# Autodesk Inventor assembly: ЛЦМК000002.00.05.00.00.00 Компактный вариант крепления
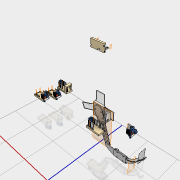
[picture p0: Inventor's stored thumbnail of the model, 180x180]
Saved by Autodesk Inventor 2021.2 (Build 252289000, 289)
## iProperties
Created: 2025-11-11
Part Number: ЛЦМК000002.00.05.00.00.00 Компактный вариант крепления
Document SubType Name: Assembly
Designer: Захаров
Author: Захаров
## Documents named in this file (17)
- C:\Users\User\Documents\CaseARHead1\ЛЦМК000002.00.05.00.00.00 Компактный вариант крепления.iam
- ЛЦМК000002.00.03.00.00.00 Облегченный вариант крепления.iam
- C:\Users\User\Documents\CaseARHead1\ЛЦМК000002.00.00.00.00.08-01.ipt
- C:\Users\User\Documents\CaseARHead1\ЛЦМК000002.00.00.00.00.15.ipt
- C:\Users\User\Documents\CaseARHead1\ЛЦМК000002.00.00.00.00.18-01.ipt
- C:\Users\User\Documents\CaseARHead1\ЛЦМК000002.00.00.00.00.19 мост.ipt
- C:\Users\User\Documents\Inventor\Content Center Files\R2021\ru-RU\Screw A2 GOST 17473-80\Винт A2.M3-6gx6 ГОСТ 17473-80.ipt
- C:\Users\User\Documents\CaseARHead1\ЛЦМК000002.00.00.00.00.20 Платформа экрана.ipt
- C:\Users\User\Documents\CaseARHead1\ЛЦМК000002.00.00.00.00.13 OLED.ipt
- C:\Users\User\Documents\CaseARHead1\ЛЦМК000002.00.00.00.00.14 Фиксатор OLED.ipt
- C:\Users\User\Documents\CaseARHead1\ЛЦМК000002.00.04.00.02.00 2 xiao.iam
- C:\Users\User\Documents\CaseARHead1\2xiao и компактный короб.iam
- C:\Users\User\Documents\CaseARHead1\Сборка1.iam
- C:\Users\User\Documents\CaseARHead1\ЛЦМК.00002.00.00.00.00.22 Крышка короба.ipt
- C:\Users\User\Documents\CaseARHead1\ЛЦМК.00002.00.00.00.00.22-01 Компактный короб.ipt
- C:\Users\User\Documents\CaseARHead1\ЛЦМК000002.00.05.00.02.00 2 xiao.iam
- C:\Users\User\Documents\CaseARHead1\ЛЦМК.00002.00.00.00.00.22-03 Компактный короб.ipt
## Components (17 placed, 15 different names)
1. ЛЦМК000002.00.00.00.00.08-01:1 — Вставка:1, Вставка:2
2. ЛЦМК000002.00.00.00.00.15:1 — Вставка:1, Вставка:2, Заподлицо:1, Совмещение:1, Заподлицо:2
3. ЛЦМК000002.00.00.00.00.18-01:1 — Заподлицо:1, Совмещение:1, Заподлицо:2, Вставка:3, Вставка:4
4. ЛЦМК000002.00.00.00.00.19 мост:1 — Вставка:3, Вставка:4, Заподлицо:3, Заподлицо:4, Заподлицо:5, Вставка:10, Заподлицо:7
5. ЛЦМК.00002.00.00.00.00.22-01 Компактный короб:2 — Совмещение:9, Совмещение:10, Совмещение:11, Совмещение:13, Вставка:10
6. Винт A2 ГОСТ 17473-80 M3-6gx6:1
7. ЛЦМК000002.00.00.00.00.20 Платформа экрана:1 — Заподлицо:3, Заподлицо:4, Вставка:6, Вставка:7, Вставка:8, Вставка:9
8. ЛЦМК000002.00.00.00.00.13 OLED:1 — Вставка:6, Вставка:7
9. ЛЦМК000002.00.00.00.00.14 Фиксатор OLED:1 — Вставка:8, Вставка:9
10. ЛЦМК000002.00.04.00.02.00 2 xiao:1 [sub-assembly] — Совмещение:9, Совмещение:10, Совмещение:11, Совмещение:12
11. 2xiao и компактный короб:1 [sub-assembly]
12. ЛЦМК.00002.00.00.00.00.22-01 Компактный короб:1 — Заподлицо:5, Заподлицо:6, Совмещение:14, Совмещение:15
13. Сборка1:1 [sub-assembly]
14. ЛЦМК.00002.00.00.00.00.22 Крышка короба:2 — Совмещение:12, Совмещение:13
15. Сборка1:2 [sub-assembly] — Заподлицо:6, Совмещение:14, Совмещение:15
16. ЛЦМК000002.00.05.00.02.00 2 xiao:1 [sub-assembly]
17. ЛЦМК.00002.00.00.00.00.22-03 Компактный короб:1 — Заподлицо:7
## Relationships (24: Insert 9, Mate 8, Flush 7)
- Вставка:1 [Insert]: ЛЦМК000002.00.00.00.00.08-01:1 ↔ ЛЦМК000002.00.00.00.00.15:1
- Вставка:2 [Insert]: ЛЦМК000002.00.00.00.00.08-01:1 ↔ ЛЦМК000002.00.00.00.00.15:1
- Заподлицо:1 [Flush]: ЛЦМК000002.00.00.00.00.15:1 ↔ ЛЦМК000002.00.00.00.00.18-01:1
- Совмещение:1 [Mate]: ЛЦМК000002.00.00.00.00.15:1 ↔ ЛЦМК000002.00.00.00.00.18-01:1
- Заподлицо:2 [Flush] (20 mm): ЛЦМК000002.00.00.00.00.15:1 ↔ ЛЦМК000002.00.00.00.00.18-01:1
- Вставка:3 [Insert]: ЛЦМК000002.00.00.00.00.18-01:1 ↔ ЛЦМК000002.00.00.00.00.19 мост:1
- Вставка:4 [Insert]: ЛЦМК000002.00.00.00.00.18-01:1 ↔ ЛЦМК000002.00.00.00.00.19 мост:1
- Заподлицо:3 [Flush]: ЛЦМК000002.00.00.00.00.19 мост:1 ↔ ЛЦМК000002.00.00.00.00.20 Платформа экрана:1
- Заподлицо:4 [Flush]: ЛЦМК000002.00.00.00.00.19 мост:1 ↔ ЛЦМК000002.00.00.00.00.20 Платформа экрана:1
- Вставка:6 [Insert]: ЛЦМК000002.00.00.00.00.20 Платформа экрана:1 ↔ ЛЦМК000002.00.00.00.00.13 OLED:1
- Вставка:7 [Insert]: ЛЦМК000002.00.00.00.00.20 Платформа экрана:1 ↔ ЛЦМК000002.00.00.00.00.13 OLED:1
- Вставка:8 [Insert]: ЛЦМК000002.00.00.00.00.20 Платформа экрана:1 ↔ ЛЦМК000002.00.00.00.00.14 Фиксатор OLED:1
- Вставка:9 [Insert]: ЛЦМК000002.00.00.00.00.20 Платформа экрана:1 ↔ ЛЦМК000002.00.00.00.00.14 Фиксатор OLED:1
- Заподлицо:5 [Flush]: ЛЦМК000002.00.00.00.00.19 мост:1 ↔ ЛЦМК.00002.00.00.00.00.22-01 Компактный короб:1
- Совмещение:9 [Mate]: ЛЦМК.00002.00.00.00.00.22-01 Компактный короб:2 ↔ ЛЦМК000002.00.04.00.02.00 2 xiao:1
- Совмещение:10 [Mate]: ЛЦМК.00002.00.00.00.00.22-01 Компактный короб:2 ↔ ЛЦМК000002.00.04.00.02.00 2 xiao:1
- Совмещение:11 [Mate]: ЛЦМК.00002.00.00.00.00.22-01 Компактный короб:2 ↔ ЛЦМК000002.00.04.00.02.00 2 xiao:1
- Совмещение:12 [Mate]: ЛЦМК000002.00.04.00.02.00 2 xiao:1 ↔ ЛЦМК.00002.00.00.00.00.22 Крышка короба:2
- Совмещение:13 [Mate]: ЛЦМК.00002.00.00.00.00.22-01 Компактный короб:2 ↔ ЛЦМК.00002.00.00.00.00.22 Крышка короба:2
- Вставка:10 [Insert]: ЛЦМК000002.00.00.00.00.19 мост:1 ↔ ЛЦМК.00002.00.00.00.00.22-01 Компактный короб:2
- Заподлицо:6 [Flush]: ЛЦМК.00002.00.00.00.00.22-01 Компактный короб:1 ↔ Сборка1:2
- Совмещение:14 [Mate] (-2 mm): ЛЦМК.00002.00.00.00.00.22-01 Компактный короб:1 ↔ Сборка1:2
- Совмещение:15 [Mate] (2.5 mm): ЛЦМК.00002.00.00.00.00.22-01 Компактный короб:1 ↔ Сборка1:2
- Заподлицо:7 [Flush]: ЛЦМК000002.00.00.00.00.19 мост:1 ↔ ЛЦМК.00002.00.00.00.00.22-03 Компактный короб:1
